# Autodesk Inventor assembly: Leg
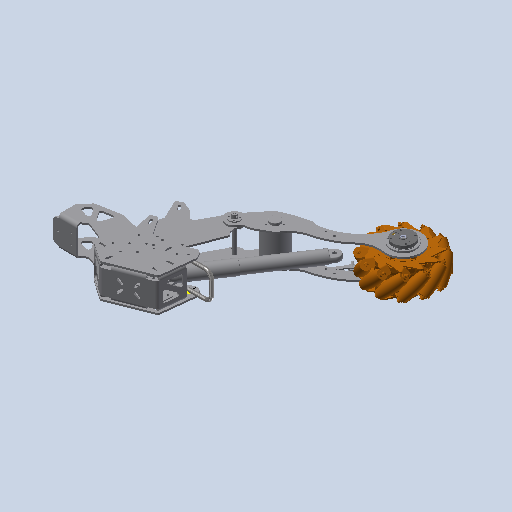
[picture p0: Inventor's stored thumbnail of the model, 512x512]
Saved by Autodesk Inventor 2025.2 (Build 292293000, 293)
## iProperties
Created: 2020-05-17
Part Number: Leg
Document SubType Name: Assembly
Designer: valer
_SolveAssemblyDoc: Frame Generator Solve Assembly
_Version: 15.0.0
Author: valer
## Documents named in this file (23)
- D:\str1ker\cad\Leg.iam
- D:\str1ker\cad\LegThigh.ipt
- D:\str1ker\cad\LegShin.ipt
- D:\str1ker\cad\LegHipSide.ipt
- D:\str1ker\cad\LegHip.ipt
- D:\str1ker\cad\LegHipFront.ipt
- D:\str1ker\cad\external\2796N15_Omni-Directional Wheel.ipt
- D:\str1ker\cad\external\MY6812-12VDC-120W-Motor.ipt
- D:\str1ker\cad\external\SprocketMDEOOSKY-25H-47T.ipt
- D:\str1ker\cad\LegHub.ipt
- D:\str1ker\cad\external\6656K234_Ultra-Thin Ball Bearing.ipt
- D:\str1ker\cad\LegInsideConnector.ipt
- D:\str1ker\cad\external\LegPotentiometer\np32hs.iam
- D:\str1ker\cad\LegHandleDesign.ipt
- D:\str1ker\cad\LegKneeShaft.ipt
- D:\str1ker\cad\external\Hub8mm.ipt
- D:\str1ker\cad\external\2920-0001-0006 assembly.iam
- D:\str1ker\cad\LegFrame\LegFrame.iam
- D:\str1ker\cad\LegChainTensioner.iam
- D:\str1ker\cad\external\WheelEncoder\am-4027 CIM_Coder_256_Encoder.iam
- D:\str1ker\cad\external\WheelEncoder\am-4027 CIM_Coder_256_Magnet.iam
- D:\str1ker\cad\external\LegActuator\ANT-38-Body.ipt
- D:\str1ker\cad\external\LegActuator\ANT-38-Shaft.ipt
## Components (30 placed, 22 different names)
1. LegThigh:1 — Flush:1, Mate:1, Mate:4, Mate:163, Mate:173, Flush:145
2. LegHipSide:1 — Flush:1, Mate:1, Mate:4, Flush:140, Flush:141, Mate:152, Mate:153, Mate:154, Angle:2, Mate:161, Mate:168, Mate:171, Mate:180
3. LegThigh:2 — Mate:133, Flush:137, Mate:136, Mate:139, Mate:145, Mate:146
4. LegHipSide:2 — Mate:145, Mate:146, Flush:140, Flush:141, Mate:156, Mate:188, Mate:200
5. MY6812-12VDC-120W-Motor:1 — Mate:77, Mate:80, Mate:89, Mate:93, Flush:4, Flush:5, Mate:132, Mate:182, Flush:146
6. LegShin:3 — Mate:77, Mate:80, Mate:163, Mate:172, Mate:175, Mate:182, Mate:184, Mate:193
7. LegShin:4 — Mate:89, Mate:132, Mate:133, Mate:139, Mate:177, Mate:183, Mate:201
8. SprocketMDEOOSKY-25H-47T:1 — Flush:4, Mate:96, Mate:110, Flush:5, Mate:181, Mate:184
9. LegHub:1 — Mate:97, Mate:108, Mate:109, Mate:110, Mate:181
10. 2796N15_Omni-Directional Wheel:1 — Mate:96, Mate:97, Mate:102, Mate:103, Mate:104, Mate:105, Mate:106, Mate:107, Mate:108, Mate:109
11. 6656K234_Ultra-Thin Ball Bearing:1 — Mate:102, Mate:183
12. 6656K234_Ultra-Thin Ball Bearing:2 — Mate:103, Mate:104
13. LegHub:3 — Mate:105, Mate:106, Mate:107, Mate:195, Mate:196, Mate:197
14. np32hs:1 [sub-assembly] — Flush:137, Mate:136, Angle:4
15. LegHandleDesign:1 — Flush:143, Mate:170, Mate:171
16. LegKneeShaft:1 — Mate:172, Mate:173, Mate:174, Mate:176, Angle:4, Flush:144, Flush:145
17. LegHip:1 — Mate:152, Mate:153, Mate:154, Mate:155, Mate:157, Mate:164, Flush:142, Mate:178
18. LegInsideConnector:5 — Mate:155, Mate:156, Mate:157, Mate:162, Mate:179
19. LegHipFront:1 — Angle:2, Mate:161, Mate:162, Mate:165
20. Hub8mm:1 — Mate:174, Mate:175, Flush:144
21. Hub8mm:2 — Mate:176, Mate:177
22. LegInsideConnector:6 — Mate:178, Mate:179, Mate:180
23. 2920-0001-0006 assembly:3 [sub-assembly] — Mate:188
24. 2920-0001-0006 assembly:4 [sub-assembly]
25. LegFrame:1 [sub-assembly]
26. LegChainTensioner:1 [sub-assembly] — Flush:146, Mate:193
27. am-4027 CIM_Coder_256_Encoder:1 [sub-assembly] — Mate:196, Mate:198
28. am-4027 CIM_Coder_256_Magnet:1 [sub-assembly] — Mate:195, Mate:197, Mate:198
29. ANT-38-Body:1 — Mate:199, Mate:200, Mate:202, Mate:203
30. ANT-38-Shaft:1 — Mate:199, Mate:201, Mate:202
## Relationships (75: Mate 61, Flush 11, Angle 3)
- Flush:1 (-5.08 mm): LegThigh:1 ↔ LegHipSide:1
- Mate:1: LegThigh:1 ↔ LegHipSide:1
- Mate:4: LegThigh:1 ↔ LegHipSide:1
- Mate:77: MY6812-12VDC-120W-Motor:1 ↔ LegShin:3
- Mate:80: MY6812-12VDC-120W-Motor:1 ↔ LegShin:3
- Mate:89: MY6812-12VDC-120W-Motor:1 ↔ LegShin:4
- Mate:93: MY6812-12VDC-120W-Motor:1
- Flush:4: MY6812-12VDC-120W-Motor:1 ↔ SprocketMDEOOSKY-25H-47T:1
- Mate:96: SprocketMDEOOSKY-25H-47T:1 ↔ 2796N15_Omni-Directional Wheel:1
- Mate:97: LegHub:1 ↔ 2796N15_Omni-Directional Wheel:1
- Mate:102: 2796N15_Omni-Directional Wheel:1 ↔ 6656K234_Ultra-Thin Ball Bearing:1
- Mate:103: 2796N15_Omni-Directional Wheel:1 ↔ 6656K234_Ultra-Thin Ball Bearing:2
- Mate:104: 2796N15_Omni-Directional Wheel:1 ↔ 6656K234_Ultra-Thin Ball Bearing:2
- Mate:105: 2796N15_Omni-Directional Wheel:1 ↔ LegHub:3
- Mate:106: 2796N15_Omni-Directional Wheel:1 ↔ LegHub:3
- Mate:107: 2796N15_Omni-Directional Wheel:1 ↔ LegHub:3
- Mate:108: LegHub:1 ↔ 2796N15_Omni-Directional Wheel:1
- Mate:109: LegHub:1 ↔ 2796N15_Omni-Directional Wheel:1
- Mate:110: SprocketMDEOOSKY-25H-47T:1 ↔ LegHub:1
- Flush:5: MY6812-12VDC-120W-Motor:1 ↔ SprocketMDEOOSKY-25H-47T:1
- Mate:132: MY6812-12VDC-120W-Motor:1 ↔ LegShin:4
- Mate:133: LegThigh:2 ↔ LegShin:4
- Flush:137: LegThigh:2 ↔ np32hs:1
- Mate:136: LegThigh:2 ↔ np32hs:1
- Mate:139: LegThigh:2 ↔ LegShin:4
- Mate:145: LegThigh:2 ↔ LegHipSide:2
- Mate:146: LegThigh:2 ↔ LegHipSide:2
- Flush:140: LegHipSide:1 ↔ LegHipSide:2
- Flush:141: LegHipSide:1 ↔ LegHipSide:2
- Mate:152: LegHipSide:1 ↔ LegHip:1
- Mate:153: LegHipSide:1 ↔ LegHip:1
- Mate:154: LegHipSide:1 ↔ LegHip:1
- Mate:155: LegHip:1 ↔ LegInsideConnector:5
- Mate:156: LegHipSide:2 ↔ LegInsideConnector:5
- Mate:157: LegHip:1 ↔ LegInsideConnector:5
- Angle:2 (0 deg): LegHipSide:1 ↔ LegHipFront:1
- Mate:161: LegHipSide:1 ↔ LegHipFront:1
- Mate:162: LegInsideConnector:5 ↔ LegHipFront:1
- Mate:163: LegThigh:1 ↔ LegShin:3
- Mate:164: LegHip:1
- Mate:165: LegHipFront:1
- Flush:142: LegHip:1
- Mate:168: LegHipSide:1
- Angle:3 (0 deg)
- Flush:143: LegHandleDesign:1
- Mate:170: LegHandleDesign:1
- Mate:171: LegHipSide:1 ↔ LegHandleDesign:1
- Mate:172: LegShin:3 ↔ LegKneeShaft:1
- Mate:173: LegThigh:1 ↔ LegKneeShaft:1
- Mate:174: LegKneeShaft:1 ↔ Hub8mm:1
- Mate:175: LegShin:3 ↔ Hub8mm:1
- Mate:176: LegKneeShaft:1 ↔ Hub8mm:2
- Mate:177: LegShin:4 ↔ Hub8mm:2
- Angle:4 (180 deg): np32hs:1 ↔ LegKneeShaft:1
- Flush:144: LegKneeShaft:1 ↔ Hub8mm:1
- Flush:145 (0.5 mm): LegThigh:1 ↔ LegKneeShaft:1
- Mate:178: LegHip:1 ↔ LegInsideConnector:6
- Mate:179: LegInsideConnector:5 ↔ LegInsideConnector:6
- Mate:180: LegHipSide:1 ↔ LegInsideConnector:6
- Mate:181: SprocketMDEOOSKY-25H-47T:1 ↔ LegHub:1
- Mate:182: MY6812-12VDC-120W-Motor:1 ↔ LegShin:3
- Mate:183: LegShin:4 ↔ 6656K234_Ultra-Thin Ball Bearing:1
- Mate:184: LegShin:3 ↔ SprocketMDEOOSKY-25H-47T:1
- Mate:188: LegHipSide:2 ↔ 2920-0001-0006 assembly:3
- Flush:146: MY6812-12VDC-120W-Motor:1 ↔ LegChainTensioner:1
- Mate:193: LegShin:3 ↔ LegChainTensioner:1
- Mate:195: LegHub:3 ↔ am-4027 CIM_Coder_256_Magnet:1
- Mate:196: LegHub:3 ↔ am-4027 CIM_Coder_256_Encoder:1
- Mate:197: LegHub:3 ↔ am-4027 CIM_Coder_256_Magnet:1
- Mate:198: am-4027 CIM_Coder_256_Encoder:1 ↔ am-4027 CIM_Coder_256_Magnet:1
- Mate:199: ANT-38-Body:1 ↔ ANT-38-Shaft:1
- Mate:200: LegHipSide:2 ↔ ANT-38-Body:1
- Mate:201: LegShin:4 ↔ ANT-38-Shaft:1
- Mate:202: ANT-38-Body:1 ↔ ANT-38-Shaft:1
- Mate:203: ANT-38-Body:1
